# Autodesk Inventor assembly: LER_intake
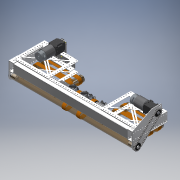
[picture p0: Inventor's stored thumbnail of the model, 180x180]
Saved by Autodesk Inventor 2019 (Build 230136000, 136)
## iProperties
Created: 2018-10-31
Part Number: LER_intake
Document SubType Name: Assembly
Designer: woodk
Author: woodk
Revision Number: ANY
## Documents named in this file (34)
- E:\Shooter1678\Workspaces\Workspace\LER_intake.iam
- E:\Shooter1678\Workspaces\Workspace\sprocket_16t_.5.ipt
- E:\Shooter1678\Workspaces\Workspace\bearing_fr8_.5hex.ipt
- E:\Shooter1678\Workspaces\Workspace\1678-16-P-0509.ipt
- E:\Shooter1678\Workspaces\Workspace\1678-16-P-0512.ipt
- E:\Shooter1678\Workspaces\Workspace\1678-16-P-0528.ipt
- E:\Shooter1678\Workspaces\Workspace\bearing_fr6_.375.ipt
- E:\Shooter1678\Workspaces\Workspace\1678-16-P-0550.ipt
- E:\Shooter1678\Workspaces\Workspace\1678-16-P-0504.ipt
- E:\Shooter1678\Workspaces\Workspace\1678-16-P-0505.ipt
- E:\Shooter1678\Workspaces\Workspace\1678-16-P-0510.ipt
- E:\Shooter1678\Workspaces\Workspace\1678-16-P-0511.ipt
- E:\Shooter1678\Workspaces\Workspace\1678-16-P-0530.ipt
- E:\Shooter1678\Workspaces\Workspace\1678-16-P-0506.ipt
- E:\Shooter1678\Workspaces\Workspace\bearing_fr8_.5.ipt
- E:\Shooter1678\Workspaces\Workspace\1678-16-P-0551.ipt
- E:\Shooter1678\Workspaces\Workspace\wheel_mecanum_4in.ipt
- E:\Shooter1678\Workspaces\Workspace\versa_planetary_10-1_775pro.iam
- E:\Shooter1678\Workspaces\Workspace\intake_chain_2.iam
- E:\Shooter1678\Workspaces\Workspace\Polycord.ipt
- E:\Shooter1678\Workspaces\Workspace\Intake front outer.ipt
- E:\Shooter1678\Workspaces\Workspace\Intake front inner.ipt
- E:\Shooter1678\Workspaces\Workspace\intake side outer.ipt
- E:\Shooter1678\Workspaces\Workspace\Intake side inner.ipt
- E:\Shooter1678\Workspaces\Workspace\Intake back outer.ipt
- E:\Shooter1678\Workspaces\Workspace\wheel_mecanum_4in_MIR.ipt
- E:\Shooter1678\Workspaces\Workspace\1678-16-P-0508.ipt
- E:\Shooter1678\Workspaces\Workspace\1678-16-P-0531.ipt
- E:\Shooter1678\Workspaces\Workspace\1678-16-P-0507.ipt
- E:\Shooter1678\Workspaces\Workspace\1678-16-P-0527.ipt
- E:\Shooter1678\Workspaces\Workspace\intake_chain.iam
- E:\Shooter1678\Workspaces\Workspace\Short Polycord.ipt
- E:\Shooter1678\Workspaces\Workspace\Mecanum bracket.ipt
- E:\Shooter1678\Workspaces\Workspace\Mecanum bracket mirror.ipt
## Components (70 placed, 58 different names)
1. 1678-16-P-0502_237 — Insert:9, Insert:10, Insert:20, Insert:95, Insert:96
2. 1678-16-P-0502_238 — Insert:5, Insert:14, Insert:91, Insert:92
3. 1678-16-P-0503_239 — Insert:15, Insert:16, Insert:21, Insert:22
4. 1678-16-P-0503_242 — Insert:11, Insert:12, Insert:27, Insert:28
5. 1678-16-P-0528_248 — Insert:7, Insert:8, Insert:9, Insert:10, Insert:11, Insert:12
6. 1678-16-P-0528_249 — Insert:19, Insert:20
7. 1678-16-P-0501_253 — Insert:1, Insert:2, Insert:6, Insert:7, Insert:8, Insert:13, Insert:17, Insert:18, Insert:19, Insert:23, Insert:24, Insert:49, Insert:50, Insert:51, Insert:52, Insert:63, Insert:64
8. 1678-16-P-0534_255 — Insert:33, Insert:49, Insert:50, Insert:53
9. bearing_fr6_.375_256 — Insert:53, Insert:61
10. 1678-16-P-0550_257 — Insert:55, Insert:61, Insert:70
11. 1678-16-P-0504_258 — Insert:21, Insert:22
12. 1678-16-P-0504_259 — Insert:23, Insert:24, Insert:29
13. 1678-16-P-0505_260 — Insert:42, Insert:47, Mate:13, Mate:14, Mate:15
14. 1678-16-P-0510_261 — Insert:37, Insert:40
15. 1678-16-P-0511_262 — Insert:38, Insert:39, Mate:10, Mate:11, Mate:12
16. 1678-16-P-0530_263 — Insert:43, Insert:62
17. 1678-16-P-0506_264 — Insert:27, Insert:28, Insert:41, Mate:7, Mate:8, Mate:9
18. 1678-16-P-0510_265 — Insert:29, Insert:32
19. 1678-16-P-0511_266 — Insert:30, Insert:31, Mate:19, Mate:20, Mate:21
20. 1678-16-P-0511_267 — Insert:34, Insert:35, Mate:16, Mate:17, Mate:18
21. 1678-16-P-0510_268 — Insert:33, Insert:36
22. bearing_fr8_.5_269 — Insert:30
23. bearing_fr8_.5_270 — Insert:31, Insert:32, Tangent:4, Tangent:5, Tangent:6
24. bearing_fr8_.5_271 — Insert:35
25. bearing_fr8_.5_272 — Insert:38
26. bearing_fr8_.5_273 — Insert:39, Insert:40
27. bearing_fr8_.5_274 — Insert:34, Insert:36
28. bearing_fr8_.5_275 — Insert:43, Insert:47, Tangent:1, Tangent:2, Tangent:3
29. 1678-16-P-0512_276 — Insert:44, Insert:45
30. bearing_fr8_.5hex_277 — Insert:41
31. 1678-16-P-0509_278 — Insert:42, Insert:44
32. sprocket_16t_.5_279 — Insert:45
33. 1678-16-P-0551_280 — Insert:59, Insert:60, Insert:89
34. 1678-16-P-0551_281 — Insert:69, Insert:71, Insert:90
35. wheel_mecanum_4in_283 — Insert:55, Insert:60
36. wheel_mecanum_4in_286 — Insert:59
37. versa_planetary_10-1_775pro_293 [sub-assembly] — Insert:48, Mate:7, Mate:8, Mate:9
38. sprocket_16t_.5_295 — Insert:48
39. intake_chain_2_296 [sub-assembly]
40. Mirror1678-16-P-0534_297 — Insert:37, Insert:51, Insert:52, Insert:54
41. bearing_fr6_.375_298 — Insert:54
42. 1678-16-P-0504:3 — Insert:1, Insert:2, Insert:62
43. 1678-16-P-0528:3 — Insert:17, Insert:18
44. 1678-16-P-0528:4 — Insert:5, Insert:6, Insert:13, Insert:14, Insert:15, Insert:16
45. Polycord:1 — Mate:12, Mate:14, Tangent:2
46. Polycord:2 — Mate:11, Mate:13, Tangent:3
47. Polycord:3 — Mate:18, Mate:19, Tangent:6
48. Polycord:4 — Mate:17, Mate:20, Tangent:5
49. Polycord:5 — Mate:16, Mate:21, Tangent:4
50. Polycord:6 — Mate:10, Mate:15, Tangent:1
51. Intake front inner:2 — Insert:63, Insert:64
52. Intake side inner:1 — Insert:95, Insert:96, Insert:97, Insert:98
53. Intake side inner:2 — Mate:22, Insert:91, Insert:92, Insert:93, Insert:94
54. wheel_mecanum_4in_MIR:1 — Insert:69
55. wheel_mecanum_4in_MIR:2 — Insert:70, Insert:71
56. bearing_fr8_.5hex:4 — Insert:81
57. bearing_fr8_.5hex:5 — Insert:74, Insert:88
58. 1678-16-P-0508:1 — Insert:76, Insert:77, Mate:27, Mate:28
59. 1678-16-P-0509:4 — Insert:76, Insert:78
60. 1678-16-P-0509:5 — Insert:77, Insert:79
61. 1678-16-P-0512:3 — Insert:78, Insert:82
62. 1678-16-P-0531:1 — Insert:79, Insert:88
63. 1678-16-P-0507:1 — Insert:74, Insert:97, Insert:98
64. sprocket_16t_.5:5 — Insert:82, Tangent:8
65. versa_planetary_10-1_775pro:2 [sub-assembly] — Mate:23, Mate:24, Mate:25
66. sprocket_16t_.5:6 — Tangent:7
67. 1678-16-P-0527:1 — Mate:22, Mate:23, Mate:24, Mate:25, Insert:81, Mate:26, Insert:93, Insert:94
68. intake_chain:1 [sub-assembly] — Mate:26, Tangent:7, Tangent:8
69. Short Polycord:1 — Insert:89, Mate:27
70. Short Polycord:2 — Insert:90, Mate:28
## Relationships (108: Insert 78, Mate 22, Tangent 8)
- Insert:1: 1678-16-P-0501_253 ↔ 1678-16-P-0504:3
- Insert:2: 1678-16-P-0501_253 ↔ 1678-16-P-0504:3
- Insert:5: 1678-16-P-0502_238 ↔ 1678-16-P-0528:4
- Insert:6: 1678-16-P-0501_253 ↔ 1678-16-P-0528:4
- Insert:7: 1678-16-P-0528_248 ↔ 1678-16-P-0501_253
- Insert:8: 1678-16-P-0528_248 ↔ 1678-16-P-0501_253
- Insert:9: 1678-16-P-0502_237 ↔ 1678-16-P-0528_248
- Insert:10: 1678-16-P-0502_237 ↔ 1678-16-P-0528_248
- Insert:11: 1678-16-P-0503_242 ↔ 1678-16-P-0528_248
- Insert:12: 1678-16-P-0503_242 ↔ 1678-16-P-0528_248
- Insert:13: 1678-16-P-0501_253 ↔ 1678-16-P-0528:4
- Insert:14: 1678-16-P-0502_238 ↔ 1678-16-P-0528:4
- Insert:15: 1678-16-P-0503_239 ↔ 1678-16-P-0528:4
- Insert:16: 1678-16-P-0503_239 ↔ 1678-16-P-0528:4
- Insert:17: 1678-16-P-0501_253 ↔ 1678-16-P-0528:3
- Insert:18: 1678-16-P-0501_253 ↔ 1678-16-P-0528:3
- Insert:19: 1678-16-P-0528_249 ↔ 1678-16-P-0501_253
- Insert:20: 1678-16-P-0502_237 ↔ 1678-16-P-0528_249
- Insert:21: 1678-16-P-0503_239 ↔ 1678-16-P-0504_258
- Insert:22: 1678-16-P-0503_239 ↔ 1678-16-P-0504_258
- Insert:23: 1678-16-P-0501_253 ↔ 1678-16-P-0504_259
- Insert:24: 1678-16-P-0501_253 ↔ 1678-16-P-0504_259
- Insert:27: 1678-16-P-0503_242 ↔ 1678-16-P-0506_264
- Insert:28: 1678-16-P-0503_242 ↔ 1678-16-P-0506_264
- Insert:29: 1678-16-P-0504_259 ↔ 1678-16-P-0510_265
- Insert:30: 1678-16-P-0511_266 ↔ bearing_fr8_.5_269
- Insert:31: 1678-16-P-0511_266 ↔ bearing_fr8_.5_270
- Insert:32 (1.5875 mm): 1678-16-P-0510_265 ↔ bearing_fr8_.5_270
- Insert:33: 1678-16-P-0534_255 ↔ 1678-16-P-0510_268
- Insert:34: 1678-16-P-0511_267 ↔ bearing_fr8_.5_274
- Insert:35: 1678-16-P-0511_267 ↔ bearing_fr8_.5_271
- Insert:36 (1.5875 mm): 1678-16-P-0510_268 ↔ bearing_fr8_.5_274
- Insert:37: 1678-16-P-0510_261 ↔ Mirror1678-16-P-0534_297
- Insert:38: 1678-16-P-0511_262 ↔ bearing_fr8_.5_272
- Insert:39: 1678-16-P-0511_262 ↔ bearing_fr8_.5_273
- Insert:40 (1.5875 mm): 1678-16-P-0510_261 ↔ bearing_fr8_.5_273
- Insert:41: 1678-16-P-0506_264 ↔ bearing_fr8_.5hex_277
- Insert:42: 1678-16-P-0505_260 ↔ 1678-16-P-0509_278
- Insert:43: 1678-16-P-0530_263 ↔ bearing_fr8_.5_275
- Insert:44: 1678-16-P-0512_276 ↔ 1678-16-P-0509_278
- Insert:45: 1678-16-P-0512_276 ↔ sprocket_16t_.5_279
- Insert:47: 1678-16-P-0505_260 ↔ bearing_fr8_.5_275
- Insert:48: versa_planetary_10-1_775pro_293 ↔ sprocket_16t_.5_295
- Mate:7: 1678-16-P-0506_264 ↔ versa_planetary_10-1_775pro_293
- Mate:8: 1678-16-P-0506_264 ↔ versa_planetary_10-1_775pro_293
- Mate:9: 1678-16-P-0506_264 ↔ versa_planetary_10-1_775pro_293
- Insert:49: 1678-16-P-0501_253 ↔ 1678-16-P-0534_255
- Insert:50: 1678-16-P-0501_253 ↔ 1678-16-P-0534_255
- Insert:51: 1678-16-P-0501_253 ↔ Mirror1678-16-P-0534_297
- Insert:52: 1678-16-P-0501_253 ↔ Mirror1678-16-P-0534_297
- Insert:53: 1678-16-P-0534_255 ↔ bearing_fr6_.375_256
- Insert:54: Mirror1678-16-P-0534_297 ↔ bearing_fr6_.375_298
- Insert:55: 1678-16-P-0550_257 ↔ wheel_mecanum_4in_283
- Insert:59: 1678-16-P-0551_280 ↔ wheel_mecanum_4in_286
- Insert:60 (15.875 mm): 1678-16-P-0551_280 ↔ wheel_mecanum_4in_283
- Insert:61 (-0.0127 mm): bearing_fr6_.375_256 ↔ 1678-16-P-0550_257
- Insert:62: 1678-16-P-0530_263 ↔ 1678-16-P-0504:3
- Mate:10: 1678-16-P-0511_262 ↔ Polycord:6
- Mate:11: 1678-16-P-0511_262 ↔ Polycord:2
- Mate:12: 1678-16-P-0511_262 ↔ Polycord:1
- Mate:13: 1678-16-P-0505_260 ↔ Polycord:2
- Mate:14: 1678-16-P-0505_260 ↔ Polycord:1
- Mate:15: 1678-16-P-0505_260 ↔ Polycord:6
- Mate:16: 1678-16-P-0511_267 ↔ Polycord:5
- Mate:17: 1678-16-P-0511_267 ↔ Polycord:4
- Mate:18: 1678-16-P-0511_267 ↔ Polycord:3
- Mate:19: 1678-16-P-0511_266 ↔ Polycord:3
- Mate:20: 1678-16-P-0511_266 ↔ Polycord:4
- Mate:21: 1678-16-P-0511_266 ↔ Polycord:5
- Tangent:1 (25.4 mm): bearing_fr8_.5_275 ↔ Polycord:6
- Tangent:2 (69.85 mm): bearing_fr8_.5_275 ↔ Polycord:1
- Tangent:3 (114.3 mm): bearing_fr8_.5_275 ↔ Polycord:2
- Tangent:4 (114.3 mm): bearing_fr8_.5_270 ↔ Polycord:5
- Tangent:5 (69.85 mm): bearing_fr8_.5_270 ↔ Polycord:4
- Tangent:6 (25.4 mm): bearing_fr8_.5_270 ↔ Polycord:3
- Insert:63: 1678-16-P-0501_253 ↔ Intake front inner:2
- Insert:64: 1678-16-P-0501_253 ↔ Intake front inner:2
- Insert:69: 1678-16-P-0551_281 ↔ wheel_mecanum_4in_MIR:1
- Insert:70: 1678-16-P-0550_257 ↔ wheel_mecanum_4in_MIR:2
- Insert:71 (15.875 mm): 1678-16-P-0551_281 ↔ wheel_mecanum_4in_MIR:2
- [Insert]: versa_planetary_10-1_775pro:2 ↔ sprocket_16t_.5:6
- Insert:74: bearing_fr8_.5hex:5 ↔ 1678-16-P-0507:1
- Insert:76: 1678-16-P-0508:1 ↔ 1678-16-P-0509:4
- Insert:77: 1678-16-P-0508:1 ↔ 1678-16-P-0509:5
- Insert:78: 1678-16-P-0509:4 ↔ 1678-16-P-0512:3
- Insert:79: 1678-16-P-0509:5 ↔ 1678-16-P-0531:1
- Mate:22: Intake side inner:2 ↔ 1678-16-P-0527:1
- Mate:23: versa_planetary_10-1_775pro:2 ↔ 1678-16-P-0527:1
- Mate:24: versa_planetary_10-1_775pro:2 ↔ 1678-16-P-0527:1
- Mate:25: versa_planetary_10-1_775pro:2 ↔ 1678-16-P-0527:1
- Insert:81: bearing_fr8_.5hex:4 ↔ 1678-16-P-0527:1
- Insert:82: 1678-16-P-0512:3 ↔ sprocket_16t_.5:5
- Mate:26 (4.9085 mm): 1678-16-P-0527:1 ↔ intake_chain:1
- Tangent:7: sprocket_16t_.5:6 ↔ intake_chain:1
- Tangent:8: sprocket_16t_.5:5 ↔ intake_chain:1
- Insert:88: bearing_fr8_.5hex:5 ↔ 1678-16-P-0531:1
- Insert:89 (1.651 mm): 1678-16-P-0551_280 ↔ Short Polycord:1
- Insert:90 (-1.651 mm): 1678-16-P-0551_281 ↔ Short Polycord:2
- Mate:27: 1678-16-P-0508:1 ↔ Short Polycord:1
- Mate:28: 1678-16-P-0508:1 ↔ Short Polycord:2
- Insert:91: 1678-16-P-0502_238 ↔ Intake side inner:2
- Insert:92: 1678-16-P-0502_238 ↔ Intake side inner:2
- Insert:93: Intake side inner:2 ↔ 1678-16-P-0527:1
- Insert:94: Intake side inner:2 ↔ 1678-16-P-0527:1
- Insert:95: 1678-16-P-0502_237 ↔ Intake side inner:1
- Insert:96: 1678-16-P-0502_237 ↔ Intake side inner:1
- Insert:97: Intake side inner:1 ↔ 1678-16-P-0507:1
- Insert:98: Intake side inner:1 ↔ 1678-16-P-0507:1
## Named parameters: d101_d53 = 0 mm
